# Autodesk Inventor assembly: ping_assembly
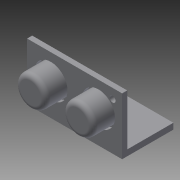
[picture p0: Inventor's stored thumbnail of the model, 180x180]
Saved by Autodesk Inventor 2015 (Build 190159000, 159)
## iProperties
Created: 2014-10-29
Part Number: ping_assembly
Document SubType Name: Assembly
Designer: Colin
Author: Colin
## Documents named in this file (3)
- E:\Users\Colin\Documents\college\marc\MicroMouse\ping_assembly.iam
- E:\Users\Colin\Documents\college\marc\MicroMouse\ping_bracket.ipt
- E:\Users\Colin\Documents\college\marc\MicroMouse\ping.ipt
## Components (2 placed, 2 different names)
1. ping_bracket:1 — Mate:1, Mate:2, Mate:3
2. ping:1 — Mate:1, Mate:2, Mate:3
## Relationships (3: Mate 3)
- Mate:1: ping_bracket:1 ↔ ping:1
- Mate:2: ping_bracket:1 ↔ ping:1
- Mate:3: ping_bracket:1 ↔ ping:1
